# Autodesk Inventor assembly: Temp_controller_demo_ASSY
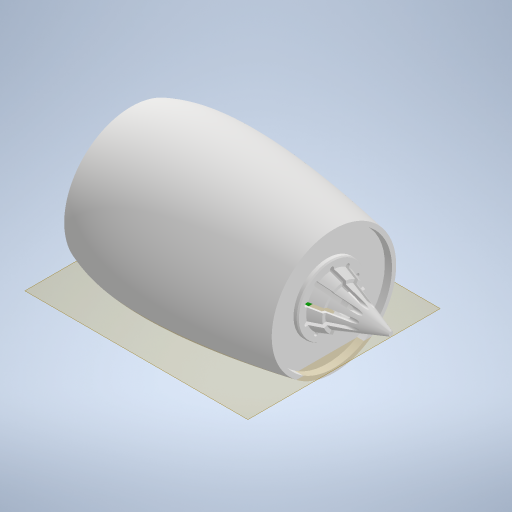
[picture p0: Inventor's stored thumbnail of the model, 512x512]
Saved by Autodesk Inventor 2024 (Build 280153000, 153)
## iProperties
Created: 2026-04-14
Part Number: Temp_controller_demo_ASSY
Document SubType Name: Assembly
Designer: Péter
Author: Péter
## Documents named in this file (4)
- D:\Inventor\Repositories\Temperature-Controller\Temp_controller_demo_ASSY.iam
- D:\Inventor\Repositories\Temperature-Controller\Import\Altium\Rack Temperature & Fan Controller_Step_Rev.1.0._2026-04-14\Rack Temperature & Fan Controller_Step_Rev.1.0._2026-04-14.ipt
- D:\Inventor\Repositories\Temperature-Controller\Temp_controller_trent.ipt
- D:\Inventor\Repositories\Temperature-Controller\Temp_controller_trent_back.ipt
## Components (3 placed, 3 different names)
1. Rack Temperature & Fan Controller_Step_Rev.1.0._2026-04-14:1 — Insert:1, Insert:2, Insert:3, Insert:4
2. Temp_controller_trent:1 — Mate:1
3. Temp_controller_trent_back:1 — Insert:1, Insert:2, Insert:3, Insert:4, Mate:1
## Relationships (5: Insert 4, Mate 1)
- Insert:1: Rack Temperature & Fan Controller_Step_Rev.1.0._2026-04-14:1 ↔ Temp_controller_trent_back:1
- Insert:2: Rack Temperature & Fan Controller_Step_Rev.1.0._2026-04-14:1 ↔ Temp_controller_trent_back:1
- Insert:3: Rack Temperature & Fan Controller_Step_Rev.1.0._2026-04-14:1 ↔ Temp_controller_trent_back:1
- Insert:4: Rack Temperature & Fan Controller_Step_Rev.1.0._2026-04-14:1 ↔ Temp_controller_trent_back:1
- Mate:1: Temp_controller_trent:1 ↔ Temp_controller_trent_back:1
